# Autodesk Inventor assembly: Chassis
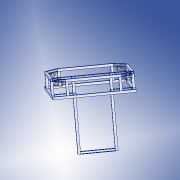
[picture p0: Inventor's stored thumbnail of the model, 180x180]
Saved by Autodesk Inventor 2017 (Build 210142000, 142)
## iProperties
Created: 2017-06-13
Part Number: Chassis
Document SubType Name: Assembly
Designer: zallen
Mass: 2624.68 g
Surface Area: 12822.9 cm^2
Volume: 1698.76 cm^3
Density: 1.54505 g/cm^3
Author: zallen
## Documents named in this file (10)
- C:\Users\zallen\Documents\GitHub\cr-laundry-robot\src\Base 2\Chassis\Chassis.iam
- C:\Users\zallen\Documents\GitHub\cr-laundry-robot\src\Base 2\Chassis\C001.ipt
- C:\Users\zallen\Documents\GitHub\cr-laundry-robot\src\Base 2\Chassis\C002.ipt
- C:\Users\zallen\Documents\GitHub\cr-laundry-robot\src\Base 2\Chassis\C003.ipt
- C:\Users\zallen\Documents\GitHub\cr-laundry-robot\src\Base 2\Chassis\C005.ipt
- C:\Users\zallen\Documents\GitHub\cr-laundry-robot\src\Base 2\Chassis\C006.ipt
- C:\Users\zallen\Documents\GitHub\cr-laundry-robot\src\Base 2\Chassis\C007.ipt
- C:\Users\zallen\Documents\GitHub\cr-laundry-robot\src\Base 2\Chassis\C008.ipt
- C:\Users\zallen\Documents\GitHub\cr-laundry-robot\src\Base 2\Chassis\C010.ipt
- C:\Users\zallen\Documents\GitHub\cr-laundry-robot\src\Base 2\Chassis\C009.ipt
## Components (36 placed, 9 different names)
1. C001:1 — Mate:2, Mate:3, Mate:10, Mate:11, Mate:67, Mate:69, Mate:70
2. C001:2 — Mate:4, Mate:5, Mate:12, Mate:13, Mate:64, Mate:65, Mate:137, Mate:140
3. C002:1 — Mate:2, Mate:3, Mate:6, Mate:7, Mate:100, Mate:101, Mate:102
4. C002:2 — Mate:4, Mate:5, Mate:8, Mate:9, Mate:66, Mate:76, Mate:97, Mate:98, Mate:99
5. C003:1 — Mate:6, Mate:7, Mate:8, Mate:9, Mate:75, Mate:77, Mate:78, Mate:135
6. C002:3 — Mate:10, Mate:11, Mate:68, Mate:74, Mate:106, Mate:107, Mate:108
7. C002:4 — Mate:12, Mate:13, Mate:14, Mate:17, Mate:60, Mate:61, Mate:62, Mate:63, Mate:103, Mate:104, Mate:105
8. C003:2 — Mate:14, Mate:17, Mate:60, Mate:61, Mate:62, Mate:71, Mate:72, Mate:73, Mate:130
9. C005:1 — Mate:106, Mate:107, Mate:108
10. C005:2 — Mate:103, Mate:104, Mate:105
11. C005:3 — Mate:100, Mate:101, Mate:102
12. C005:4 — Mate:97, Mate:98, Mate:99
13. C006:1 — Mate:63, Mate:64
14. C006:2 — Mate:65, Mate:66, Mate:87, Mate:88
15. C006:3 — Mate:67, Mate:68
16. C006:4 — Mate:69, Mate:70, Mate:89, Mate:90
17. C006:5 — Mate:71, Mate:72
18. C006:6 — Mate:73, Mate:74, Mate:94
19. C006:7 — Mate:75, Mate:76, Mate:91
20. C006:8 — Mate:77, Mate:78
21. C007:1 — Mate:87, Mate:88, Mate:92, Mate:96, Mate:118, Mate:119, Mate:120, Mate:121
22. C007:2 — Mate:89, Mate:90, Mate:95
23. C008:1 — Mate:91, Mate:92, Mate:128
24. C008:2 — Mate:94, Mate:95, Mate:96, Mate:125
25. C008:3 — Mate:109, Mate:110, Mate:113, Mate:115, Mate:117, Mate:124, Mate:131, Mate:132, Mate:136, Mate:138
26. C008:4 — Mate:111, Mate:112, Mate:114, Mate:116, Mate:122, Mate:123, Mate:127, Mate:133, Mate:134, Mate:139, Mate:141
27. C010:1 — Mate:109, Mate:110, Mate:111, Mate:112
28. C010:2 — Mate:113, Mate:114, Mate:115, Mate:116
29. C006:9 — Mate:117, Mate:118, Mate:119, Mate:126
30. C006:10 — Mate:120, Mate:121, Mate:122, Mate:123, Mate:129
31. C009:1 — Mate:124, Mate:125, Mate:126
32. C009:2 — Mate:127, Mate:128, Mate:129
33. C009:3 — Mate:130, Mate:131, Mate:132
34. C009:4 — Mate:133, Mate:134, Mate:135
35. C006:11 — Mate:136, Mate:137, Mate:138
36. C006:12 — Mate:139, Mate:140, Mate:141
## Relationships (87: Mate 87)
- Mate:2: C001:1 ↔ C002:1
- Mate:3: C001:1 ↔ C002:1
- Mate:4: C001:2 ↔ C002:2
- Mate:5: C001:2 ↔ C002:2
- Mate:6: C002:1 ↔ C003:1
- Mate:7: C002:1 ↔ C003:1
- Mate:8: C002:2 ↔ C003:1
- Mate:9: C002:2 ↔ C003:1
- Mate:10: C001:1 ↔ C002:3
- Mate:11: C001:1 ↔ C002:3
- Mate:12: C001:2 ↔ C002:4
- Mate:13: C001:2 ↔ C002:4
- Mate:14: C002:4 ↔ C003:2
- Mate:17: C002:4 ↔ C003:2
- Mate:60: C002:4 ↔ C003:2
- Mate:61: C002:4 ↔ C003:2
- Mate:62: C002:4 ↔ C003:2
- Mate:63: C002:4 ↔ C006:1
- Mate:64: C001:2 ↔ C006:1
- Mate:65: C001:2 ↔ C006:2
- Mate:66: C002:2 ↔ C006:2
- Mate:67: C001:1 ↔ C006:3
- Mate:68: C002:3 ↔ C006:3
- Mate:69: C001:1 ↔ C006:4
- Mate:70: C001:1 ↔ C006:4
- Mate:71: C003:2 ↔ C006:5
- Mate:72: C003:2 ↔ C006:5
- Mate:73: C003:2 ↔ C006:6
- Mate:74: C002:3 ↔ C006:6
- Mate:75: C003:1 ↔ C006:7
- Mate:76: C002:2 ↔ C006:7
- Mate:77: C003:1 ↔ C006:8
- Mate:78: C003:1 ↔ C006:8
- Mate:87: C006:2 ↔ C007:1
- Mate:88: C006:2 ↔ C007:1
- Mate:89: C006:4 ↔ C007:2
- Mate:90: C006:4 ↔ C007:2
- Mate:91: C006:7 ↔ C008:1
- Mate:92: C007:1 ↔ C008:1
- Mate:94: C006:6 ↔ C008:2
- Mate:95: C007:2 ↔ C008:2
- Mate:96: C007:1 ↔ C008:2
- Mate:97: C002:2 ↔ C005:4
- Mate:98: C002:2 ↔ C005:4
- Mate:99: C002:2 ↔ C005:4
- Mate:100: C002:1 ↔ C005:3
- Mate:101: C002:1 ↔ C005:3
- Mate:102: C002:1 ↔ C005:3
- Mate:103: C002:4 ↔ C005:2
- Mate:104: C002:4 ↔ C005:2
- Mate:105: C002:4 ↔ C005:2
- Mate:106: C002:3 ↔ C005:1
- Mate:107: C002:3 ↔ C005:1
- Mate:108: C002:3 ↔ C005:1
- Mate:109: C008:3 ↔ C010:1
- Mate:110: C008:3 ↔ C010:1
- Mate:111: C008:4 ↔ C010:1
- Mate:112: C008:4 ↔ C010:1
- Mate:113: C008:3 ↔ C010:2
- Mate:114: C008:4 ↔ C010:2
- Mate:115: C008:3 ↔ C010:2
- Mate:116: C008:4 ↔ C010:2
- Mate:117: C008:3 ↔ C006:9
- Mate:118: C007:1 ↔ C006:9
- Mate:119: C007:1 ↔ C006:9
- Mate:120: C007:1 ↔ C006:10
- Mate:121: C007:1 ↔ C006:10
- Mate:122: C008:4 ↔ C006:10
- Mate:123: C008:4 ↔ C006:10
- Mate:124: C008:3 ↔ C009:1
- Mate:125: C008:2 ↔ C009:1
- Mate:126: C006:9 ↔ C009:1
- Mate:127: C008:4 ↔ C009:2
- Mate:128: C008:1 ↔ C009:2
- Mate:129: C006:10 ↔ C009:2
- Mate:130: C003:2 ↔ C009:3
- Mate:131: C008:3 ↔ C009:3
- Mate:132: C008:3 ↔ C009:3
- Mate:133: C008:4 ↔ C009:4
- Mate:134: C008:4 ↔ C009:4
- Mate:135: C003:1 ↔ C009:4
- Mate:136: C008:3 ↔ C006:11
- Mate:137: C001:2 ↔ C006:11
- Mate:138: C008:3 ↔ C006:11
- Mate:139: C008:4 ↔ C006:12
- Mate:140: C001:2 ↔ C006:12
- Mate:141: C008:4 ↔ C006:12
